# Autodesk Inventor assembly: PaddleCollection2.1.ipt
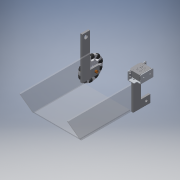
[picture p0: Inventor's stored thumbnail of the model, 180x180]
Saved by Autodesk Inventor 2019 (Build 230136000, 136)
## iProperties
Created: 2018-10-20
Part Number: PaddleCollection2.1.ipt
Document SubType Name: Assembly
Designer: User
Author: User
## Documents named in this file (12)
- C:\Robotics\CAD\2018-19_CAD\Collection\PaddleCollection2.1.ipt.iam
- C:\Robotics\CAD\2018-19_CAD\Collection\PaddleCollection2.1AxleSupport.ipt
- C:\Robotics\CAD\2018-19_CAD\Collection\PaddleCollection2.1Casing.ipt
- C:\Robotics\CAD\2018-19_CAD\Collection\PaddleCollectionFloor.ipt
- C:\Robotics\CAD\COTSParts\Tetrix\Tetrix Wheel 3 in omni.ipt
- C:\Robotics\CAD\COTSParts\Tetrix\Bronze bushing.ipt
- C:\Robotics\CAD\COTSParts\Tetrix\Tetrix shaft collar.ipt
- C:\Robotics\CAD\COTSParts\Tetrix\Tetrix Hub - axle.ipt
- C:\Robotics\CAD\COTSParts\Rev\REV-41-1097SmartServo.ipt
- C:\Robotics\CAD\COTSParts\Tetrix\39060_txm-standard servo bracket.ipt
- C:\Robotics\CAD\COTSParts\Tetrix\Tetrix bracket - angle.ipt
- C:\Robotics\CAD\2018-19_CAD\Collection\PaddleCollection2.1ServoSupport.ipt
## Components (13 placed, 11 different names)
1. PaddleCollection2.1AxleSupport:1 — Mate:1, Mate:2, Flush:1, Insert:1
2. PaddleCollection2.1Casing:1 — Flush:3, Mate:5, Mate:6, Mate:1
3. PaddleCollection2.1Casing:2 — Mate:3, Mate:4, Flush:2, Flush:4, Mate:8, Flush:5
4. PaddleCollectionFloor:1 — Mate:2, Flush:1, Mate:3, Mate:4, Flush:2, Flush:3, Mate:5, Mate:6
5. Tetrix Wheel 3 in omni:1 — Insert:3, Insert:4
6. Bronze bushing:1 — Insert:1, Insert:2
7. Bronze bushing:2 — Insert:5
8. Tetrix shaft collar:1 — Insert:2, Insert:3
9. Tetrix Hub - axle:1 — Insert:4, Insert:5
10. REV-41-1097SmartServo:1 — Insert:6, Angle:1
11. 39060_txm-standard servo bracket:1 — Insert:6, Angle:1, Insert:7, Insert:8
12. Tetrix bracket - angle:1 — Insert:7, Insert:8, Insert:9, Angle:2
13. PaddleCollection2.1ServoSupport:1 — Flush:4, Mate:8, Flush:5, Insert:9, Angle:2
## Relationships (23: Insert 9, Mate 7, Flush 5, Angle 2)
- Mate:1: PaddleCollection2.1AxleSupport:1 ↔ PaddleCollection2.1Casing:1
- Mate:2: PaddleCollection2.1AxleSupport:1 ↔ PaddleCollectionFloor:1
- Flush:1: PaddleCollection2.1AxleSupport:1 ↔ PaddleCollectionFloor:1
- Mate:3: PaddleCollection2.1Casing:2 ↔ PaddleCollectionFloor:1
- Mate:4: PaddleCollection2.1Casing:2 ↔ PaddleCollectionFloor:1
- Flush:2: PaddleCollection2.1Casing:2 ↔ PaddleCollectionFloor:1
- Flush:3: PaddleCollection2.1Casing:1 ↔ PaddleCollectionFloor:1
- Mate:5: PaddleCollection2.1Casing:1 ↔ PaddleCollectionFloor:1
- Mate:6: PaddleCollection2.1Casing:1 ↔ PaddleCollectionFloor:1
- Insert:1: PaddleCollection2.1AxleSupport:1 ↔ Bronze bushing:1
- Insert:2: Bronze bushing:1 ↔ Tetrix shaft collar:1
- Insert:3: Tetrix Wheel 3 in omni:1 ↔ Tetrix shaft collar:1
- Insert:4: Tetrix Wheel 3 in omni:1 ↔ Tetrix Hub - axle:1
- Insert:5: Bronze bushing:2 ↔ Tetrix Hub - axle:1
- Insert:6: REV-41-1097SmartServo:1 ↔ 39060_txm-standard servo bracket:1
- Angle:1 (0 deg): REV-41-1097SmartServo:1 ↔ 39060_txm-standard servo bracket:1
- Insert:7: 39060_txm-standard servo bracket:1 ↔ Tetrix bracket - angle:1
- Insert:8: 39060_txm-standard servo bracket:1 ↔ Tetrix bracket - angle:1
- Flush:4: PaddleCollection2.1Casing:2 ↔ PaddleCollection2.1ServoSupport:1
- Mate:8: PaddleCollection2.1Casing:2 ↔ PaddleCollection2.1ServoSupport:1
- Flush:5: PaddleCollection2.1Casing:2 ↔ PaddleCollection2.1ServoSupport:1
- Insert:9: Tetrix bracket - angle:1 ↔ PaddleCollection2.1ServoSupport:1
- Angle:2 (0 deg): Tetrix bracket - angle:1 ↔ PaddleCollection2.1ServoSupport:1
